# Autodesk Inventor assembly: final assembly
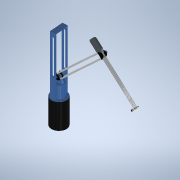
[picture p0: Inventor's stored thumbnail of the model, 180x180]
Saved by Autodesk Inventor 2020 (Build 240168000, 168)
## iProperties
Created: 2020-07-11
Part Number: final assembly
Document SubType Name: Assembly
Designer: Vikki
Mass: 4.14366e+06 g
Surface Area: 369331 cm^2
Volume: 4.00043e+06 cm^3
Density: 1.0358 g/cm^3
Author: Vikki
## Documents named in this file (8)
- D:\projects\Intelligent Picking\vicky models\articulated arm\final assembly.iam
- E:\project inventor pro\flipkart grid models\cartisian bot\workoutlook.2.ipt
- D:\projects\Intelligent Picking\vicky models\articulated arm\2  link z rotate.ipt
- D:\projects\Intelligent Picking\vicky models\articulated arm\base fix.ipt
- D:\projects\Intelligent Picking\vicky models\articulated arm\arm j2 assemny.iam
- D:\projects\Intelligent Picking\vicky models\articulated arm\arm j3 assembly.iam
- D:\projects\Intelligent Picking\vicky models\articulated arm\arm j4 assembly.iam
- E:\project inventor pro\flipkart grid models\cartisian bot 2\universal end effector.ipt
## Components (7 placed, 7 different names)
1. workoutlook.2:1 — Mate:2, Flush:1, Flush:4, Mate:4, Mate:5, Mate:8, Angle:2, Flush:12, Angle:4, Angle:7, Angle:8
2. 2  link z rotate:1 — Mate:6, Mate:7, Mate:14, Flush:11, Angle:7
3. base fix:1 — Flush:4, Mate:4, Mate:5, Mate:6, Mate:7, Mate:15, Flush:13
4. arm j2 assemny:1 [sub-assembly] — Mate:12, Flush:9, Mate:14, Flush:11, Angle:5, Angle:8
5. arm j4 assembly:1 [sub-assembly] — Mate:11, Angle:1, Flush:7, Flush:8, Mate:13, Flush:10, Angle:6
6. universal end effector:1 — Mate:11, Angle:1, Flush:7, Flush:8, Angle:2, Flush:12
7. arm j3 assembly:2 [sub-assembly] — Mate:12, Flush:9, Mate:13, Flush:10, Angle:4, Angle:5, Angle:6
## Relationships (27: Mate 11, Flush 9, Angle 7)
- Mate:2: workoutlook.2:1
- Flush:1: workoutlook.2:1
- Flush:4: workoutlook.2:1 ↔ base fix:1
- Mate:4 (2300 mm): workoutlook.2:1 ↔ base fix:1
- Mate:5 (-500 mm): workoutlook.2:1 ↔ base fix:1
- Mate:6: 2  link z rotate:1 ↔ base fix:1
- Mate:7: 2  link z rotate:1 ↔ base fix:1
- Mate:8: workoutlook.2:1
- Mate:11: arm j4 assembly:1 ↔ universal end effector:1
- Angle:1 (90 deg): arm j4 assembly:1 ↔ universal end effector:1
- Flush:7 (25 mm): arm j4 assembly:1 ↔ universal end effector:1
- Flush:8 (30 mm): arm j4 assembly:1 ↔ universal end effector:1
- Mate:12: arm j2 assemny:1 ↔ arm j3 assembly:2
- Flush:9 (35 mm): arm j2 assemny:1 ↔ arm j3 assembly:2
- Mate:13: arm j4 assembly:1 ↔ arm j3 assembly:2
- Flush:10 (-25 mm): arm j4 assembly:1 ↔ arm j3 assembly:2
- Mate:14: 2  link z rotate:1 ↔ arm j2 assemny:1
- Flush:11 (-15 mm): 2  link z rotate:1 ↔ arm j2 assemny:1
- Angle:2 (0 deg): workoutlook.2:1 ↔ universal end effector:1
- Flush:12: workoutlook.2:1 ↔ universal end effector:1
- Angle:4 (180 deg): workoutlook.2:1 ↔ arm j3 assembly:2
- Angle:5 (0 deg): arm j2 assemny:1 ↔ arm j3 assembly:2
- Angle:6 (0 deg): arm j4 assembly:1 ↔ arm j3 assembly:2
- Angle:7 (180 deg): workoutlook.2:1 ↔ 2  link z rotate:1
- Angle:8 (180 deg): workoutlook.2:1 ↔ arm j2 assemny:1
- Mate:15: base fix:1
- Flush:13: base fix:1
